# Autodesk Inventor assembly: SuperBlock US
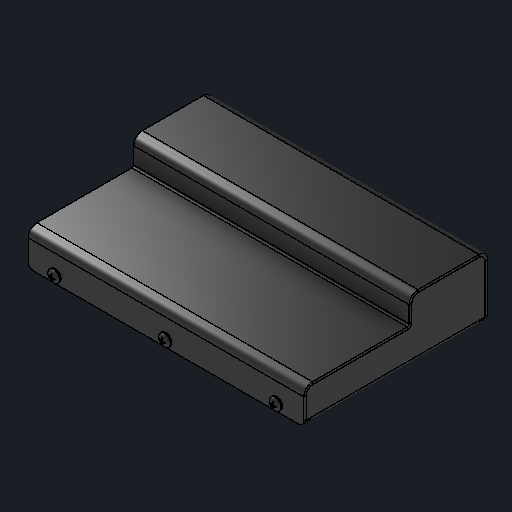
[picture p0: Inventor's stored thumbnail of the model, 512x512]
Saved by Autodesk Inventor 2026.2 (Build 302298000, 298)
## iProperties
Created: 2026-06-19
Part Number: SuperBlock US
Document SubType Name: Assembly
Designer: JoshuaEah
Author: JoshuaEah
## Documents named in this file (6)
- C:\Users\JoshuaEah\Documents\GitHub\Designed-Trinkets\Guitar\Modular Pedalboard\Pedals\SuperBlock US\SuperBlock US.iam
- C:\Users\JoshuaEah\Documents\GitHub\Designed-Trinkets\Guitar\Modular Pedalboard\Pedals\SuperBlock US\Top Shell.ipt
- C:\Users\JoshuaEah\Documents\GitHub\Designed-Trinkets\Guitar\Modular Pedalboard\Pedals\SuperBlock US\Bottom Shell.ipt
- C:\Users\JoshuaEah\Documents\GitHub\Designed-Trinkets\Guitar\Modular Pedalboard\Pedals\SuperBlock US\TS Input Jack.ipt
- C:\Users\JoshuaEah\Documents\GitHub\Designed-Trinkets\Guitar\Modular Pedalboard\Pedals\SuperBlock US\6-32x0.25 PN PH2.ipt
- C:\Users\JoshuaEah\Documents\GitHub\Designed-Trinkets\Guitar\Modular Pedalboard\Pedals\SuperBlock US\DC Jack.ipt
## Components (17 placed, 6 different names)
1. Bottom Shell:1 — Insert:1, Insert:2, Insert:7, Insert:8, Mate:5, Mate:6
2. Top Shell:1 — Mate:3, Mate:4, Insert:3, Insert:4, Insert:1, Insert:2
3. TS Output Jack:5 — Mate:5, Mate:6
4. TS Input Jack:1 — Mate:3, Mate:4
5. TS Input Jack:2
6. TS Input Jack:3
7. TS Input Jack:4
8. 6-32x0.25 PN PH2:1 — Insert:3
9. 6-32x0.25 PN PH2:2
10. 6-32x0.25 PN PH2:3
11. 6-32x0.25 PN PH2:4 — Insert:4
12. 6-32x0.25 PN PH2:5
13. 6-32x0.25 PN PH2:6
14. DC Jack:1 — Insert:7
15. DC Jack:2
16. 6-32x0.25 PN PH2:7 — Insert:8
17. 6-32x0.25 PN PH2:8
## Component patterns: 1/4" TS Jacks (4 elements), Front Mounting Screws (3 elements), Rear Mounting Screws (3 elements), DC Input Jacks (2 elements), Left Mounting Screws (2 elements)
## Relationships (10: Insert 6, Mate 4)
- Mate:3: Top Shell:1 ↔ TS Input Jack:1
- Mate:4: Top Shell:1 ↔ TS Input Jack:1
- Insert:3: Top Shell:1 ↔ 6-32x0.25 PN PH2:1
- Insert:4: Top Shell:1 ↔ 6-32x0.25 PN PH2:4
- Insert:1: Bottom Shell:1 ↔ Top Shell:1
- Insert:2: Bottom Shell:1 ↔ Top Shell:1
- Insert:7: Bottom Shell:1 ↔ DC Jack:1
- Insert:8: Bottom Shell:1 ↔ 6-32x0.25 PN PH2:7
- Mate:5: Bottom Shell:1 ↔ TS Output Jack:5
- Mate:6: Bottom Shell:1 ↔ TS Output Jack:5
